# Autodesk Inventor assembly: AssemblyV2
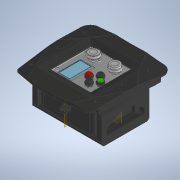
[picture p0: Inventor's stored thumbnail of the model, 180x180]
Saved by Autodesk Inventor 2022 (Build 260153000, 153)
## iProperties
Created: 2020-11-05
Part Number: AssemblyV2
Document SubType Name: Assembly
Designer: Viktor
Author: Viktor
## Documents named in this file (22)
- C:\Users\Viktor\Documents\GitHub\MARV-Hardware-Mechanical\InventorProjects\OCU - Operator Control Unit\OCU_Assembly.iam
- C:\Users\Viktor\Documents\GitHub\MARV-Hardware-Mechanical\InventorProjects\OCU - Operator Control Unit\Button\107283268-9-xb4_bl42\xb4_bl42.iam
- C:\Users\Viktor\Documents\GitHub\MARV-Hardware-Mechanical\InventorProjects\OCU - Operator Control Unit\Button\107283650-9-xb4_bw36b5\xb4_ba21.iam
- C:\Users\Viktor\Documents\GitHub\MARV-Hardware-Mechanical\InventorProjects\OCU - Operator Control Unit\Connector\c-dt15-4p-99-3d.ipt
- C:\Users\Viktor\Documents\GitHub\MARV-Hardware-Mechanical\InventorProjects\OCU - Operator Control Unit\Connector\dt15-2p-p010.ipt
- C:\Users\Viktor\Documents\GitHub\MARV-Hardware-Mechanical\InventorProjects\OCU - Operator Control Unit\Connector\c-dt15-6p-99-3d.ipt
- C:\Users\Viktor\Documents\GitHub\MARV-Hardware-Mechanical\InventorProjects\OCU - Operator Control Unit\Box\96023234_B-141309-PC-V0-G-7024.iam
- C:\Users\Viktor\Documents\GitHub\MARV-Hardware-Mechanical\InventorProjects\OCU - Operator Control Unit\Other\Adafruit_2719.ipt
- C:\Users\Viktor\Documents\GitHub\MARV-Hardware-Mechanical\InventorProjects\OCU - Operator Control Unit\Button\imp7Z432.ipt
- C:\Users\Viktor\Documents\GitHub\MARV-Hardware-Mechanical\InventorProjects\OCU - Operator Control Unit\Button\imp7Z462.ipt
- C:\Users\Viktor\Documents\GitHub\MARV-Hardware-Mechanical\InventorProjects\OCU - Operator Control Unit\Other\AssemblyPlate.ipt
- C:\Users\Viktor\Documents\GitHub\MARV-Hardware-Mechanical\InventorProjects\OCU - Operator Control Unit\Screws\Spacer8mm_m3_970080354.ipt
- C:\Users\Viktor\Documents\GitHub\MARV-Hardware-Mechanical\InventorProjects\OCU - Operator Control Unit\Other\OCU_PCB.ipt
- C:\Users\Viktor\Documents\GitHub\MARV-Hardware-Mechanical\InventorProjects\OCU - Operator Control Unit\Holder\BottomHolder.ipt
- C:\Users\Viktor\Documents\GitHub\MARV-Hardware-Mechanical\InventorProjects\OCU - Operator Control Unit\Other\WaveRunner_GloveBox.ipt
- C:\Users\Viktor\Documents\GitHub\MARV-Hardware-Mechanical\InventorProjects\OCU - Operator Control Unit\Holder\SideHolder.ipt
- C:\Users\Viktor\Documents\GitHub\MARV-Hardware-Mechanical\InventorProjects\OCU - Operator Control Unit\Screws\pop_PSZROX-0315.ipt
- C:\Users\Viktor\Documents\GitHub\MARV-Hardware-Mechanical\InventorProjects\OCU - Operator Control Unit\Holder\TopHolder.ipt
- C:\Users\Viktor\Documents\GitHub\MARV-Hardware-Mechanical\InventorProjects\OCU - Operator Control Unit\Holder\SideHolder_MIR.ipt
- C:\Users\Viktor\Documents\GitHub\MARV-Hardware-Mechanical\InventorProjects\OCU - Operator Control Unit\Other\SprayPaint.ipt
- C:\Users\Viktor\Documents\GitHub\MARV-Hardware-Mechanical\InventorProjects\OCU - Operator Control Unit\Connector\px0443\px0443.iam
- C:\Users\Viktor\Documents\GitHub\MARV-Hardware-Mechanical\InventorProjects\OCU - Operator Control Unit\Button\imp7Z422.ipt
## Components (39 placed, 21 different names)
1. 96023234_B-141309-PC-V0-G-7024:1 [sub-assembly] — Mate:1, Mate:2, Mate:3, Mate:4, Rigid:7, Rigid:8, Rigid:9, Mate:5, Flush:5, Flush:6, Mate:6, Rigid:13, Rigid:30, Flush:7, Rigid:35, Rigid:36, Rigid:37, Rigid:38, Rigid:39
2. xb4_ba21:1 [sub-assembly] — Rigid:7
3. xb4_bl42:1 [sub-assembly] — Rigid:8
4. c-dt15-4p-99-3d:1 — Mate:1, Flush:1, Flush:3, Mate:6
5. dt15-2p-p010:1 — Mate:2, Flush:2, Flush:3
6. c-dt15-6p-99-3d:1 — Mate:4, Flush:2, Flush:4, Flush:5
7. c-dt15-6p-99-3d:2 — Mate:3, Flush:1, Flush:4, Mate:5, Flush:6
8. Adafruit_2719:1 — Rigid:9
9. imp7Z432:1 — Rigid:38
10. imp7Z462:1 — Rigid:37
11. AssemblyPlate:1 — Rigid:13, Rigid:14, Rigid:15, Rigid:16, Rigid:17, Rigid:18, Rigid:19, Rigid:20, Rigid:21, Rigid:22, Rigid:23, Rigid:24, Rigid:25, Rigid:26, Rigid:27, Rigid:28
12. Spacer8mm_m3_970080354:1 — Rigid:18
13. Spacer8mm_m3_970080354:2 — Rigid:19
14. Spacer8mm_m3_970080354:3 — Rigid:20
15. Spacer8mm_m3_970080354:4 — Rigid:21
16. Spacer8mm_m3_970080354:5 — Rigid:23
17. Spacer8mm_m3_970080354:6 — Rigid:24
18. Spacer8mm_m3_970080354:7 — Rigid:22
19. Spacer8mm_m3_970080354:8 — Rigid:17
20. Spacer8mm_m3_970080354:9 — Rigid:16
21. Spacer8mm_m3_970080354:10 — Rigid:15, Rigid:29
22. Spacer8mm_m3_970080354:11 — Rigid:14
23. Spacer8mm_m3_970080354:12 — Rigid:28
24. Spacer8mm_m3_970080354:13 — Rigid:27
25. Spacer8mm_m3_970080354:14 — Rigid:26
26. Spacer8mm_m3_970080354:15 — Rigid:25
27. OCU_PCB:1 — Rigid:29
28. BottomHolder:1 — Rigid:30, Rigid:31
29. WaveRunner_GloveBox:1 — Flush:7
30. SideHolder:1 — Rigid:31, Rigid:32, Rigid:33, Rigid:34, Angle:1
31. pop_PSZROX-0315:1 — Rigid:32, Insert:1
32. pop_PSZROX-0315:2 — Rigid:34
33. pop_PSZROX-0315:3 — Rigid:33
34. TopHolder:1 — Insert:1, Angle:1
35. SideHolder_MIR:1
36. SprayPaint:1
37. px0443:1 [sub-assembly] — Rigid:35
38. imp7Z422:1 — Rigid:39
39. imp7Z422:2 — Rigid:36
## Relationships (45: WeldJoint 30, Flush 7, Mate 6, Insert 1, Angle 1)
- Mate:1: 96023234_B-141309-PC-V0-G-7024:1 ↔ c-dt15-4p-99-3d:1
- Mate:2: 96023234_B-141309-PC-V0-G-7024:1 ↔ dt15-2p-p010:1
- Mate:3: 96023234_B-141309-PC-V0-G-7024:1 ↔ c-dt15-6p-99-3d:2
- Mate:4: 96023234_B-141309-PC-V0-G-7024:1 ↔ c-dt15-6p-99-3d:1
- Rigid:7 [WeldJoint]: 96023234_B-141309-PC-V0-G-7024:1 ↔ xb4_ba21:1
- Rigid:8 [WeldJoint]: 96023234_B-141309-PC-V0-G-7024:1 ↔ xb4_bl42:1
- Rigid:9 [WeldJoint] (-3 mm): 96023234_B-141309-PC-V0-G-7024:1 ↔ Adafruit_2719:1
- Flush:1: c-dt15-4p-99-3d:1 ↔ c-dt15-6p-99-3d:2
- Flush:2: dt15-2p-p010:1 ↔ c-dt15-6p-99-3d:1
- Flush:3: c-dt15-4p-99-3d:1 ↔ dt15-2p-p010:1
- Flush:4: c-dt15-6p-99-3d:1 ↔ c-dt15-6p-99-3d:2
- Mate:5 (5 mm): 96023234_B-141309-PC-V0-G-7024:1 ↔ c-dt15-6p-99-3d:2
- Flush:5 (-5 mm): 96023234_B-141309-PC-V0-G-7024:1 ↔ c-dt15-6p-99-3d:1
- Flush:6 (3 mm): 96023234_B-141309-PC-V0-G-7024:1 ↔ c-dt15-6p-99-3d:2
- Mate:6 (5 mm): 96023234_B-141309-PC-V0-G-7024:1 ↔ c-dt15-4p-99-3d:1
- Rigid:13 [WeldJoint]: 96023234_B-141309-PC-V0-G-7024:1 ↔ AssemblyPlate:1
- Rigid:14 [WeldJoint]: AssemblyPlate:1 ↔ Spacer8mm_m3_970080354:11
- Rigid:15 [WeldJoint]: AssemblyPlate:1 ↔ Spacer8mm_m3_970080354:10
- Rigid:16 [WeldJoint]: AssemblyPlate:1 ↔ Spacer8mm_m3_970080354:9
- Rigid:17 [WeldJoint]: AssemblyPlate:1 ↔ Spacer8mm_m3_970080354:8
- Rigid:18 [WeldJoint]: AssemblyPlate:1 ↔ Spacer8mm_m3_970080354:1
- Rigid:19 [WeldJoint]: AssemblyPlate:1 ↔ Spacer8mm_m3_970080354:2
- Rigid:20 [WeldJoint]: AssemblyPlate:1 ↔ Spacer8mm_m3_970080354:3
- Rigid:21 [WeldJoint]: AssemblyPlate:1 ↔ Spacer8mm_m3_970080354:4
- Rigid:22 [WeldJoint]: AssemblyPlate:1 ↔ Spacer8mm_m3_970080354:7
- Rigid:23 [WeldJoint]: AssemblyPlate:1 ↔ Spacer8mm_m3_970080354:5
- Rigid:24 [WeldJoint]: AssemblyPlate:1 ↔ Spacer8mm_m3_970080354:6
- Rigid:25 [WeldJoint]: AssemblyPlate:1 ↔ Spacer8mm_m3_970080354:15
- Rigid:26 [WeldJoint]: AssemblyPlate:1 ↔ Spacer8mm_m3_970080354:14
- Rigid:27 [WeldJoint]: AssemblyPlate:1 ↔ Spacer8mm_m3_970080354:13
- Rigid:28 [WeldJoint]: AssemblyPlate:1 ↔ Spacer8mm_m3_970080354:12
- Rigid:29 [WeldJoint]: Spacer8mm_m3_970080354:10 ↔ OCU_PCB:1
- Rigid:30 [WeldJoint]: 96023234_B-141309-PC-V0-G-7024:1 ↔ BottomHolder:1
- Flush:7 (2 mm): 96023234_B-141309-PC-V0-G-7024:1 ↔ WaveRunner_GloveBox:1
- Rigid:31 [WeldJoint]: BottomHolder:1 ↔ SideHolder:1
- Rigid:32 [WeldJoint]: SideHolder:1 ↔ pop_PSZROX-0315:1
- Rigid:33 [WeldJoint]: SideHolder:1 ↔ pop_PSZROX-0315:3
- Rigid:34 [WeldJoint]: SideHolder:1 ↔ pop_PSZROX-0315:2
- Insert:1: pop_PSZROX-0315:1 ↔ TopHolder:1
- Angle:1 (0 deg): SideHolder:1 ↔ TopHolder:1
- Rigid:35 [WeldJoint]: 96023234_B-141309-PC-V0-G-7024:1 ↔ px0443:1
- Rigid:36 [WeldJoint]: 96023234_B-141309-PC-V0-G-7024:1 ↔ imp7Z422:2
- Rigid:37 [WeldJoint]: 96023234_B-141309-PC-V0-G-7024:1 ↔ imp7Z462:1
- Rigid:38 [WeldJoint]: 96023234_B-141309-PC-V0-G-7024:1 ↔ imp7Z432:1
- Rigid:39 [WeldJoint]: 96023234_B-141309-PC-V0-G-7024:1 ↔ imp7Z422:1
